# Autodesk Inventor assembly: Ceiling Comp 2
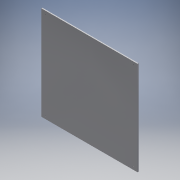
[picture p0: Inventor's stored thumbnail of the model, 180x180]
Saved by Autodesk Inventor 2017 (Build 210142000, 142)
## iProperties
Created: 2017-05-26
Part Number: Ceiling Comp 2
Document SubType Name: Assembly
Designer: cas7
Author: cas7
## Documents named in this file (3)
- C:\Users\Public\Documents\Autodesk\.desktop-connect\.docstore\guided-tutorial-plugin\INVNTOR\Compartment Modeling\Ceiling Comp 2.iam
- C:\Users\Public\Documents\Autodesk\.desktop-connect\.docstore\guided-tutorial-plugin\INVNTOR\Compartment Modeling\7x56.25 Gyp.ipt
- C:\Users\Public\Documents\Autodesk\.desktop-connect\.docstore\guided-tutorial-plugin\INVNTOR\Compartment Modeling\56.25x48 Gyp Top.ipt
## Components (2 placed, 2 different names)
1. 7x56.25 Gyp:1 — Mate:1, Mate:2
2. 56.25x48 Gyp Top:1 — Mate:1, Mate:2
## Relationships (2: Mate 2)
- Mate:1: 7x56.25 Gyp:1 ↔ 56.25x48 Gyp Top:1
- Mate:2: 7x56.25 Gyp:1 ↔ 56.25x48 Gyp Top:1
